# Autodesk Inventor assembly: phalanx
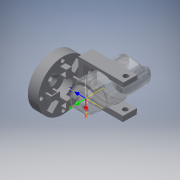
[picture p0: Inventor's stored thumbnail of the model, 180x180]
Saved by Autodesk Inventor 2019 (Build 230136000, 136)
## iProperties
Created: 2024-05-02
Part Number: phalanx
Material: Generisch
Document SubType Name: Assembly
Designer: nic
Author: nic
## Documents named in this file (4)
- C:\Users\Nicolas Frick\Sync\OneDrive\wtm\nicol_rh8d\atxmega_qenc\inventor\phalanx.iam
- C:\Users\Nicolas Frick\Sync\OneDrive\wtm\nias\nias_description\inventor_files\hand\r_rh8d_refac\phalanx_refac.ipt
- C:\Users\Nicolas Frick\Sync\OneDrive\wtm\nicol_rh8d\atxmega_qenc\inventor\amt_socket.ipt
- C:\Users\Nicolas Frick\Sync\OneDrive\wtm\nias\nias_description\inventor_files\amt_dragster.ipt
## Components (3 placed, 3 different names)
1. phalanx_refac:1 — Passend:1, Fluchtend:1, Passend:2, Passend:3
2. amt_socket:1 — Passend:2, Passend:3, Passend:4, Passend:5
3. amt_dragster:1 — Passend:4, Passend:5
## Relationships (6: Mate 5, Flush 1)
- Passend:1 [Mate]: phalanx_refac:1
- Fluchtend:1 [Flush]: phalanx_refac:1
- Passend:2 [Mate]: phalanx_refac:1 ↔ amt_socket:1
- Passend:3 [Mate] (8 mm): phalanx_refac:1 ↔ amt_socket:1
- Passend:4 [Mate]: amt_socket:1 ↔ amt_dragster:1
- Passend:5 [Mate]: amt_socket:1 ↔ amt_dragster:1
